# Autodesk Inventor assembly: Top_Bevel
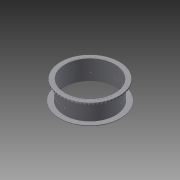
[picture p0: Inventor's stored thumbnail of the model, 180x180]
Saved by Autodesk Inventor 2015 (Build 190159000, 159)
## iProperties
Created: 2016-03-23
Part Number: Top_Bevel
Document SubType Name: Assembly
Designer: david_000
Author: david_000
## Documents named in this file (4)
- C:\Users\david_000\Documents\Drone-Git\Drone\3D Models\Project\Chasis\Top_Bevel.iam
- C:\Users\david_000\Documents\Drone-Git\Drone\3D Models\Project\Beveled_Ring.ipt
- C:\Users\david_000\Documents\Drone-Git\Drone\3D Models\Project\Chasis\Top_Bevel_Base_Top.ipt
- C:\Users\david_000\Documents\Drone-Git\Drone\3D Models\Project\Chasis\Top_Bevel_Base_Bottom.ipt
## Components (3 placed, 3 different names)
1. Top_Bevel_Base_Top:1 — Insert:1, Insert:2, Angle:1
2. Top_Bevel_Base_Bottom:1 — Insert:1, Angle:1
3. Beveled_Ring:1 — Insert:2
## Relationships (3: Insert 2, Angle 1)
- Insert:1: Top_Bevel_Base_Top:1 ↔ Top_Bevel_Base_Bottom:1
- Insert:2: Top_Bevel_Base_Top:1 ↔ Beveled_Ring:1
- Angle:1 (0 deg): Top_Bevel_Base_Top:1 ↔ Top_Bevel_Base_Bottom:1
